# Autodesk Inventor assembly: DYS SF2207 Motor
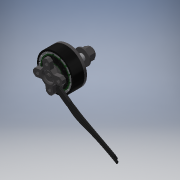
[picture p0: Inventor's stored thumbnail of the model, 180x180]
Saved by Autodesk Inventor 2019 (Build 230136000, 136)
## iProperties
Created: 2020-07-12
Part Number: DYS SF2207 Motor
Material: Ogólny
Document SubType Name: Assembly
Designer: Karol
Sending System: Autodesk Translation Framework v9.3.0.1241
Preprocessor: ST-DEVELOPER v18.1
Title: C:/Users/Olavides/Desktop/DYS SF2207 Motor/DYS SF2207 Motor.step
## Documents named in this file (2)
- C:\Users\Karol\Desktop\Koło naukowe KNMG\Drone\dys-sf2207-brushless-motor-1.snapshot.1\DYS SF2207 Motor.iam
- C:\Users\Karol\Desktop\Koło naukowe KNMG\Drone\dys-sf2207-brushless-motor-1.snapshot.1\DYS SF2207 Brushless Motor v5 (2).iam
## Components (1 placed, 1 different names)
1. DYS SF2207 Brushless Motor v5 (2):1 [sub-assembly]
## Relationships (1: Flush 1)
- Równoległy:1 [Flush] (50 mm)
